# Autodesk Inventor assembly: service_design_project_draft
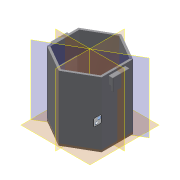
[picture p0: Inventor's stored thumbnail of the model, 180x180]
Saved by Autodesk Inventor 2017 (Build 210142000, 142)
## iProperties
Created: 2018-11-28
Part Number: service_design_project_draft
Document SubType Name: Assembly
Designer: jpb34
Author: jpb34
## Documents named in this file (10)
- C:\Users\jacob\Documents\School\College\ENGR 101C\Service Design Project\service_design_project_draft.iam
- C:\Users\jacob\Documents\School\College\ENGR 101C\Service Design Project\HEX_BASE.ipt
- C:\Users\jacob\Documents\School\College\ENGR 101C\Service Design Project\side.ipt
- C:\Users\jacob\Documents\School\College\ENGR 101C\Service Design Project\Mid_Plate.ipt
- C:\Users\jacob\Documents\School\College\ENGR 101C\Service Design Project\side_w_door.ipt
- C:\Users\jacob\Documents\School\College\ENGR 101C\Service Design Project\handle.ipt
- C:\Users\jacob\Documents\School\College\ENGR 101C\Service Design Project\mid_plate_support.ipt
- C:\Users\jacob\Documents\School\College\ENGR 101C\Service Design Project\door.ipt
- C:\Users\jacob\Documents\School\College\ENGR 101C\Service Design Project\handle_MIR1.ipt
- C:\Users\jacob\Documents\School\College\ENGR 101C\Service Design Project\Plexiglass.ipt
## Components (15 placed, 9 different names)
1. HEX_BASE:1 — Mate:1, Flush:1, Mate:2, Mate:5, Mate:8, Mate:17
2. Mid_Plate:1 — Mate:5
3. side_w_door:1 — Mate:6, Mate:7, Mate:8, Mate:9, Mate:10, Mate:11, Mate:12, Mate:13, Mate:14, Mate:18, Mate:19, Mate:20
4. handle:1 — Mate:9, Mate:10, Mate:11
5. handle_MIR1:1
6. door:1 — Mate:12, Mate:13, Mate:14
7. Plexiglass:1 — Mate:18, Mate:19, Mate:20
8. side:1 — Mate:1, Flush:1, Mate:2, Symmetry:1, Mate:7, Mate:15, Mate:16
9. side:2
10. side:3
11. side:4
12. side:5 — Mate:6
13. mid_plate_support:1 — Mate:15, Mate:16, Mate:17
14. mid_plate_support:4
15. mid_plate_support:5
## Component patterns: (5 elements, first: side:1), (3 elements, first: mid_plate_support:1)
## Relationships (22: Mate 20, Flush 1, Symmetry 1)
- Mate:1: HEX_BASE:1 ↔ side:1
- Flush:1: HEX_BASE:1 ↔ side:1
- Mate:2: HEX_BASE:1 ↔ side:1
- Symmetry:1: side:1
- Mate:3
- Mate:4
- Mate:5 (101.6 mm): HEX_BASE:1 ↔ Mid_Plate:1
- Mate:6: side_w_door:1 ↔ side:5
- Mate:7: side_w_door:1 ↔ side:1
- Mate:8: HEX_BASE:1 ↔ side_w_door:1
- Mate:9: side_w_door:1 ↔ handle:1
- Mate:10 (12.7 mm): side_w_door:1 ↔ handle:1
- Mate:11 (146.05 mm): side_w_door:1 ↔ handle:1
- Mate:12: side_w_door:1 ↔ door:1
- Mate:13: side_w_door:1 ↔ door:1
- Mate:14: side_w_door:1 ↔ door:1
- Mate:15: side:1 ↔ mid_plate_support:1
- Mate:16 (44.45 mm): side:1 ↔ mid_plate_support:1
- Mate:17: HEX_BASE:1 ↔ mid_plate_support:1
- Mate:18: side_w_door:1 ↔ Plexiglass:1
- Mate:19: side_w_door:1 ↔ Plexiglass:1
- Mate:20: side_w_door:1 ↔ Plexiglass:1
